# Autodesk Inventor assembly: Manipulator
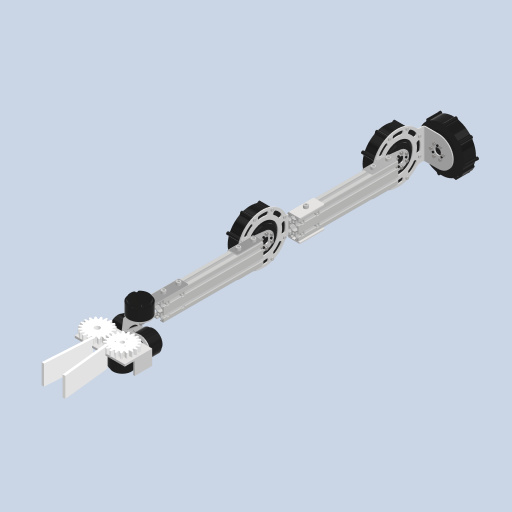
[picture p0: Inventor's stored thumbnail of the model, 512x512]
Saved by Autodesk Inventor 2023 (Build 270158000, 158)
## iProperties
Created: 2024-11-08
Part Number: Manipulator
Document SubType Name: Assembly
Designer: kiyo
Author: kiyo
## Documents named in this file (22)
- D:\GitHub\inventor\syu-si\OfficeRobot\Manipulator\Manipulator.iam
- D:\GitHub\inventor\syu-si\OfficeRobot\ReadyMade\Steadywin\GIM8108-8.iam
- D:\GitHub\inventor\syu-si\OfficeRobot\Manipulator\sholder-roll-bracket.ipt
- D:\GitHub\inventor\syu-si\OfficeRobot\Manipulator\elbow-pitch-bracket.ipt
- D:\GitHub\inventor\syu-si\OfficeRobot\Manipulator\Hand.iam
- D:\GitHub\inventor\syu-si\OfficeRobot\ReadyMade\Screw\M3_6mm.ipt
- D:\GitHub\inventor\syu-si\OfficeRobot\ReadyMade\Screw\SCB5-22.ipt
- D:\GitHub\inventor\syu-si\OfficeRobot\ReadyMade\Screw\HNTP5-5.ipt
- D:\GitHub\inventor\syu-si\OfficeRobot\Manipulator\pitch_plate_40mm.ipt
- D:\GitHub\inventor\syu-si\OfficeRobot\ReadyMade\Steadywin\GIM3505-8_with-driver.ipt
- D:\GitHub\inventor\syu-si\OfficeRobot\Manipulator\wrist_roll_plate.ipt
- D:\GitHub\inventor\syu-si\OfficeRobot\Manipulator\wrist-pitch-plate.ipt
- D:\GitHub\inventor\syu-si\OfficeRobot\Manipulator\wrist-yaw-plate.ipt
- D:\GitHub\inventor\syu-si\OfficeRobot\ReadyMade\Screw\M2-5_6mm.ipt
- D:\GitHub\inventor\syu-si\OfficeRobot\ReadyMade\Aluminum-frame\HFS5-2040-200-AV160-BV190-Z5-YA10-YB40.ipt
- D:\GitHub\inventor\syu-si\OfficeRobot\ReadyMade\Screw\SCB5-46.ipt
- D:\GitHub\inventor\syu-si\OfficeRobot\ReadyMade\Screw\SLBNR5.ipt
- D:\GitHub\inventor\syu-si\OfficeRobot\ReadyMade\Screw\CBSH3-8.ipt
- D:\GitHub\inventor\syu-si\OfficeRobot\ReadyMade\Screw\HNTT5-5.ipt
- D:\GitHub\inventor\syu-si\OfficeRobot\ReadyMade\Screw\SCB5-8.ipt
- D:\GitHub\inventor\syu-si\OfficeRobot\ReadyMade\Screw\FWSJJ-D5-V2_6-T4_5.ipt
- D:\GitHub\inventor\syu-si\OfficeRobot\ReadyMade\Screw\M2-5_10mm.ipt
## Components (108 placed, 21 different names)
1. elbow-pitch-bracket:1 — 挿入:180, 挿入:181, 挿入:234, 挿入:235, 挿入:256, 挿入:257, 挿入:268, 挿入:269, 挿入:270, 挿入:271, 挿入:272, 挿入:273, 挿入:274, 挿入:275, 挿入:295, 挿入:296, 挿入:299, 挿入:300
2. sholder-roll-bracket:1 — 挿入:1, 挿入:2, 挿入:3, 肩ヨー, 挿入:102, 挿入:103, 挿入:104, 挿入:105, 挿入:106, 挿入:107, 挿入:260, 挿入:261, 挿入:262, 挿入:263, 挿入:264, 挿入:265, 挿入:266, 挿入:267
3. pitch_plate_40mm:1 — 挿入:165, 挿入:182, 挿入:183, 挿入:184, 挿入:185, 挿入:186, 挿入:187, 挿入:232, 挿入:233, 角度:7, 挿入:250, 挿入:251, 挿入:254, 挿入:255, 挿入:278, 挿入:279, 角度:9, 角度:10
4. pitch_plate_40mm:2 — 挿入:190, 挿入:191, 挿入:192, 挿入:193, 挿入:194, 挿入:195, 挿入:196, 角度:8, 挿入:236, 挿入:237, 挿入:248, 挿入:249, 挿入:252, 挿入:253
5. wrist_roll_plate:1 — 挿入:220, 挿入:227, 挿入:228, 挿入:229, 挿入:230, 挿入:231, 挿入:283, 挿入:284, 挿入:285
6. wrist-pitch-plate:1 — 挿入:211, 挿入:212, 挿入:213, 挿入:217, 挿入:218, 挿入:219, 挿入:220, 挿入:280, 挿入:281, 挿入:282, 角度:15
7. wrist-yaw-plate:1 — 挿入:203, 挿入:204, 挿入:205, 挿入:206, 挿入:207, 挿入:211, 挿入:238, 挿入:239, 挿入:258, 挿入:259, 挿入:291, 挿入:292
8. HFS5-2040-200-AV160-BV190-Z5-YA10-YB40:1 — 挿入:232, 挿入:233, 挿入:234, 挿入:235, 挿入:246, 挿入:247, 挿入:293, 挿入:294, 角度:13, 角度:14
9. HFS5-2040-200-AV160-BV190-Z5-YA10-YB40:2 — 挿入:236, 挿入:237, 挿入:238, 挿入:239, 挿入:244, 挿入:245, 角度:11, 角度:12
10. Hand:1 [sub-assembly] — ハンド, 挿入:301
11. SCB5-22:1 — 挿入:247
12. SCB5-22:2 — 挿入:246
13. SCB5-22:3 — 挿入:244
14. SCB5-22:4 — 挿入:245
15. SCB5-46:1 — 挿入:250
16. SCB5-46:2 — 挿入:251
17. SCB5-46:3 — 挿入:248
18. SCB5-46:4 — 挿入:249
19. SLBNR5:1 — 挿入:255
20. SLBNR5:2 — 挿入:254
21. SLBNR5:3 — 挿入:252
22. SLBNR5:4 — 挿入:253
23. SLBNR5:5 — 挿入:256
24. SLBNR5:6 — 挿入:257
25. SLBNR5:7 — 挿入:258
26. SLBNR5:8 — 挿入:259
27. HNTT5-5:1 — 挿入:276, 角度:10
28. HNTT5-5:2 — 挿入:277, 角度:9
29. SCB5-8:1 — 挿入:276, 挿入:278
30. SCB5-8:2 — 挿入:277, 挿入:279
31. FWSJJ-D5-V2_6-T4_5:7 — 挿入:286
32. FWSJJ-D5-V2_6-T4_5:8 — 挿入:287
33. FWSJJ-D5-V2_6-T4_5:9 — 挿入:288
34. HNTT5-5:3 — 角度:11
35. HNTT5-5:4 — 角度:12
36. SCB5-8:3 — 挿入:291
37. SCB5-8:4 — 挿入:292
38. SCB5-22:5 — 挿入:294
39. SCB5-22:6 — 挿入:293
40. SLBNR5:9 — 挿入:296
41. SLBNR5:10 — 挿入:295
42. HNTT5-5:5 — 角度:13
43. SCB5-8:5 — 挿入:299
44. HNTT5-5:6 — 角度:14
45. SCB5-8:6 — 挿入:300
46. M3_6mm:1 — 挿入:183
47. M3_6mm:2 — 挿入:186
48. M3_6mm:3 — 挿入:187
49. M3_6mm:4 — 挿入:184
50. M3_6mm:5 — 挿入:185
51. M3_6mm:6 — 挿入:182
52. M3_6mm:7 — 挿入:192
53. M3_6mm:8 — 挿入:191
54. M3_6mm:9 — 挿入:196
55. M3_6mm:10 — 挿入:195
56. M3_6mm:11 — 挿入:194
57. M3_6mm:12 — 挿入:193
58. M3_6mm:13 — 挿入:107
59. M3_6mm:14 — 挿入:106
60. M3_6mm:15 — 挿入:105
61. M3_6mm:16 — 挿入:102
62. M3_6mm:17 — 挿入:103
63. M3_6mm:18 — 挿入:104
64. CBSH3-8:1 — 挿入:261
65. CBSH3-8:2 — 挿入:262
66. CBSH3-8:3 — 挿入:266
67. CBSH3-8:4 — 挿入:265
68. CBSH3-8:5 — 挿入:267
69. CBSH3-8:6 — 挿入:264
70. CBSH3-8:7 — 挿入:263
71. CBSH3-8:8 — 挿入:260
72. CBSH3-8:9 — 挿入:268
73. CBSH3-8:10 — 挿入:270
74. CBSH3-8:11 — 挿入:275
75. CBSH3-8:12 — 挿入:274
76. CBSH3-8:13 — 挿入:273
77. CBSH3-8:14 — 挿入:272
78. CBSH3-8:15 — 挿入:271
79. CBSH3-8:16 — 挿入:269
80. M2-5_6mm:1 — 挿入:205
81. M2-5_6mm:2 — 挿入:207
82. M2-5_6mm:3 — 挿入:206
83. M2-5_6mm:7 — 挿入:229
84. M2-5_6mm:8 — 挿入:230
85. M2-5_6mm:9 — 挿入:231
86. M2-5_6mm:4 — 挿入:217
87. M2-5_6mm:5 — 挿入:218
88. M2-5_6mm:6 — 挿入:219
89. M2-5_10mm:1
90. M2-5_10mm:2
91. M2-5_10mm:3
92. M2-5_10mm:4
93. M2-5_10mm:5
94. M2-5_10mm:6
95. FWSJJ-D5-V2_6-T4_5:1 — 挿入:280
96. FWSJJ-D5-V2_6-T4_5:2 — 挿入:282
97. FWSJJ-D5-V2_6-T4_5:3 — 挿入:281
98. FWSJJ-D5-V2_6-T4_5:4 — 挿入:283
99. FWSJJ-D5-V2_6-T4_5:5 — 挿入:285
100. FWSJJ-D5-V2_6-T4_5:6 — 挿入:284
101. HNTP5-5:7
102. HNTP5-5:8
103. GIM3505-8_with-driver:1 — 挿入:203, 挿入:204
104. GIM3505-8_with-driver:3 — 挿入:227, 挿入:228, 挿入:286, 挿入:287, 挿入:288, 角度:16, 挿入:301
105. GIM3505-8_with-driver:4 — 挿入:212, 挿入:213
106. GIM8108-8:1 [sub-assembly] — 挿入:1
107. GIM8108-8:2 [sub-assembly] — 挿入:2, 挿入:3, 挿入:165
108. GIM8108-8:3 [sub-assembly] — 挿入:180, 挿入:181, 挿入:190
## Relationships (126: Insert 114, Angle 12)
- 挿入:1 [Insert]: sholder-roll-bracket:1 ↔ GIM8108-8:1
- 挿入:2 [Insert]: sholder-roll-bracket:1 ↔ GIM8108-8:2
- 挿入:3 [Insert]: sholder-roll-bracket:1 ↔ GIM8108-8:2
- 肩ヨー [Angle] (0 deg): sholder-roll-bracket:1
- ハンド [Angle] (0 deg): Hand:1
- 挿入:102 [Insert]: sholder-roll-bracket:1 ↔ M3_6mm:16
- 挿入:103 [Insert]: sholder-roll-bracket:1 ↔ M3_6mm:17
- 挿入:104 [Insert]: sholder-roll-bracket:1 ↔ M3_6mm:18
- 挿入:105 [Insert]: sholder-roll-bracket:1 ↔ M3_6mm:15
- 挿入:106 [Insert]: sholder-roll-bracket:1 ↔ M3_6mm:14
- 挿入:107 [Insert]: sholder-roll-bracket:1 ↔ M3_6mm:13
- 挿入:165 [Insert]: pitch_plate_40mm:1 ↔ GIM8108-8:2
- 挿入:180 [Insert]: elbow-pitch-bracket:1 ↔ GIM8108-8:3
- 挿入:181 [Insert]: elbow-pitch-bracket:1 ↔ GIM8108-8:3
- 挿入:182 [Insert]: pitch_plate_40mm:1 ↔ M3_6mm:6
- 挿入:183 [Insert]: pitch_plate_40mm:1 ↔ M3_6mm:1
- 挿入:184 [Insert]: pitch_plate_40mm:1 ↔ M3_6mm:4
- 挿入:185 [Insert]: pitch_plate_40mm:1 ↔ M3_6mm:5
- 挿入:186 [Insert]: pitch_plate_40mm:1 ↔ M3_6mm:2
- 挿入:187 [Insert]: pitch_plate_40mm:1 ↔ M3_6mm:3
- 挿入:190 [Insert]: pitch_plate_40mm:2 ↔ GIM8108-8:3
- 挿入:191 [Insert]: pitch_plate_40mm:2 ↔ M3_6mm:8
- 挿入:192 [Insert]: pitch_plate_40mm:2 ↔ M3_6mm:7
- 挿入:193 [Insert]: pitch_plate_40mm:2 ↔ M3_6mm:12
- 挿入:194 [Insert]: pitch_plate_40mm:2 ↔ M3_6mm:11
- 挿入:195 [Insert]: pitch_plate_40mm:2 ↔ M3_6mm:10
- 挿入:196 [Insert]: pitch_plate_40mm:2 ↔ M3_6mm:9
- 挿入:203 [Insert]: wrist-yaw-plate:1 ↔ GIM3505-8_with-driver:1
- 挿入:204 [Insert]: wrist-yaw-plate:1 ↔ GIM3505-8_with-driver:1
- 挿入:205 [Insert]: wrist-yaw-plate:1 ↔ M2-5_6mm:1
- 挿入:206 [Insert]: wrist-yaw-plate:1 ↔ M2-5_6mm:3
- 挿入:207 [Insert]: wrist-yaw-plate:1 ↔ M2-5_6mm:2
- 挿入:211 [Insert] (3.5 mm): wrist-pitch-plate:1 ↔ wrist-yaw-plate:1
- 挿入:212 [Insert]: wrist-pitch-plate:1 ↔ GIM3505-8_with-driver:4
- 挿入:213 [Insert]: wrist-pitch-plate:1 ↔ GIM3505-8_with-driver:4
- 挿入:217 [Insert]: wrist-pitch-plate:1 ↔ M2-5_6mm:4
- 挿入:218 [Insert]: wrist-pitch-plate:1 ↔ M2-5_6mm:5
- 挿入:219 [Insert]: wrist-pitch-plate:1 ↔ M2-5_6mm:6
- 挿入:220 [Insert] (3.5 mm): wrist_roll_plate:1 ↔ wrist-pitch-plate:1
- [Insert]: wrist-pitch-plate:1 ↔ M2-5_10mm:1
- [Insert]: wrist-pitch-plate:1 ↔ M2-5_10mm:2
- [Insert]: wrist-pitch-plate:1 ↔ M2-5_10mm:3
- [Insert]: wrist_roll_plate:1 ↔ M2-5_10mm:6
- [Insert]: wrist_roll_plate:1 ↔ M2-5_10mm:4
- [Insert]: wrist_roll_plate:1 ↔ M2-5_10mm:5
- 挿入:227 [Insert]: wrist_roll_plate:1 ↔ GIM3505-8_with-driver:3
- 挿入:228 [Insert]: wrist_roll_plate:1 ↔ GIM3505-8_with-driver:3
- 挿入:229 [Insert]: wrist_roll_plate:1 ↔ M2-5_6mm:7
- 挿入:230 [Insert]: wrist_roll_plate:1 ↔ M2-5_6mm:8
- 挿入:231 [Insert]: wrist_roll_plate:1 ↔ M2-5_6mm:9
- 挿入:232 [Insert]: pitch_plate_40mm:1 ↔ HFS5-2040-200-AV160-BV190-Z5-YA10-YB40:1
- 挿入:233 [Insert]: pitch_plate_40mm:1 ↔ HFS5-2040-200-AV160-BV190-Z5-YA10-YB40:1
- 挿入:234 [Insert] (6 mm): elbow-pitch-bracket:1 ↔ HFS5-2040-200-AV160-BV190-Z5-YA10-YB40:1
- 挿入:235 [Insert] (6 mm): elbow-pitch-bracket:1 ↔ HFS5-2040-200-AV160-BV190-Z5-YA10-YB40:1
- 角度:7 [Angle] (0 deg): pitch_plate_40mm:1
- 角度:8 [Angle] (0 deg): pitch_plate_40mm:2
- 挿入:236 [Insert]: pitch_plate_40mm:2 ↔ HFS5-2040-200-AV160-BV190-Z5-YA10-YB40:2
- 挿入:237 [Insert]: pitch_plate_40mm:2 ↔ HFS5-2040-200-AV160-BV190-Z5-YA10-YB40:2
- 挿入:238 [Insert] (6 mm): wrist-yaw-plate:1 ↔ HFS5-2040-200-AV160-BV190-Z5-YA10-YB40:2
- 挿入:239 [Insert] (6 mm): wrist-yaw-plate:1 ↔ HFS5-2040-200-AV160-BV190-Z5-YA10-YB40:2
- 挿入:244 [Insert]: HFS5-2040-200-AV160-BV190-Z5-YA10-YB40:2 ↔ SCB5-22:3
- 挿入:245 [Insert]: HFS5-2040-200-AV160-BV190-Z5-YA10-YB40:2 ↔ SCB5-22:4
- 挿入:246 [Insert]: HFS5-2040-200-AV160-BV190-Z5-YA10-YB40:1 ↔ SCB5-22:2
- 挿入:247 [Insert]: HFS5-2040-200-AV160-BV190-Z5-YA10-YB40:1 ↔ SCB5-22:1
- 挿入:248 [Insert]: pitch_plate_40mm:2 ↔ SCB5-46:3
- 挿入:249 [Insert]: pitch_plate_40mm:2 ↔ SCB5-46:4
- 挿入:250 [Insert]: pitch_plate_40mm:1 ↔ SCB5-46:1
- 挿入:251 [Insert]: pitch_plate_40mm:1 ↔ SCB5-46:2
- 挿入:252 [Insert]: pitch_plate_40mm:2 ↔ SLBNR5:3
- 挿入:253 [Insert]: pitch_plate_40mm:2 ↔ SLBNR5:4
- 挿入:254 [Insert]: pitch_plate_40mm:1 ↔ SLBNR5:2
- 挿入:255 [Insert]: pitch_plate_40mm:1 ↔ SLBNR5:1
- 挿入:256 [Insert]: elbow-pitch-bracket:1 ↔ SLBNR5:5
- 挿入:257 [Insert]: elbow-pitch-bracket:1 ↔ SLBNR5:6
- 挿入:258 [Insert]: wrist-yaw-plate:1 ↔ SLBNR5:7
- 挿入:259 [Insert]: wrist-yaw-plate:1 ↔ SLBNR5:8
- 挿入:260 [Insert]: sholder-roll-bracket:1 ↔ CBSH3-8:8
- 挿入:261 [Insert]: sholder-roll-bracket:1 ↔ CBSH3-8:1
- 挿入:262 [Insert]: sholder-roll-bracket:1 ↔ CBSH3-8:2
- 挿入:263 [Insert]: sholder-roll-bracket:1 ↔ CBSH3-8:7
- 挿入:264 [Insert]: sholder-roll-bracket:1 ↔ CBSH3-8:6
- 挿入:265 [Insert]: sholder-roll-bracket:1 ↔ CBSH3-8:4
- 挿入:266 [Insert]: sholder-roll-bracket:1 ↔ CBSH3-8:3
- 挿入:267 [Insert]: sholder-roll-bracket:1 ↔ CBSH3-8:5
- 挿入:268 [Insert]: elbow-pitch-bracket:1 ↔ CBSH3-8:9
- 挿入:269 [Insert]: elbow-pitch-bracket:1 ↔ CBSH3-8:16
- 挿入:270 [Insert]: elbow-pitch-bracket:1 ↔ CBSH3-8:10
- 挿入:271 [Insert]: elbow-pitch-bracket:1 ↔ CBSH3-8:15
- 挿入:272 [Insert]: elbow-pitch-bracket:1 ↔ CBSH3-8:14
- 挿入:273 [Insert]: elbow-pitch-bracket:1 ↔ CBSH3-8:13
- 挿入:274 [Insert]: elbow-pitch-bracket:1 ↔ CBSH3-8:12
- 挿入:275 [Insert]: elbow-pitch-bracket:1 ↔ CBSH3-8:11
- 挿入:276 [Insert] (3.2 mm): HNTT5-5:1 ↔ SCB5-8:1
- 挿入:277 [Insert] (3.2 mm): HNTT5-5:2 ↔ SCB5-8:2
- 挿入:278 [Insert]: pitch_plate_40mm:1 ↔ SCB5-8:1
- 挿入:279 [Insert]: pitch_plate_40mm:1 ↔ SCB5-8:2
- 角度:9 [Angle] (0 deg): pitch_plate_40mm:1 ↔ HNTT5-5:2
- 角度:10 [Angle] (0 deg): pitch_plate_40mm:1 ↔ HNTT5-5:1
- 挿入:280 [Insert]: wrist-pitch-plate:1 ↔ FWSJJ-D5-V2_6-T4_5:1
- 挿入:281 [Insert]: wrist-pitch-plate:1 ↔ FWSJJ-D5-V2_6-T4_5:3
- 挿入:282 [Insert]: wrist-pitch-plate:1 ↔ FWSJJ-D5-V2_6-T4_5:2
- 挿入:283 [Insert]: wrist_roll_plate:1 ↔ FWSJJ-D5-V2_6-T4_5:4
- 挿入:284 [Insert]: wrist_roll_plate:1 ↔ FWSJJ-D5-V2_6-T4_5:6
- 挿入:285 [Insert]: wrist_roll_plate:1 ↔ FWSJJ-D5-V2_6-T4_5:5
- 挿入:286 [Insert]: FWSJJ-D5-V2_6-T4_5:7 ↔ GIM3505-8_with-driver:3
- 挿入:287 [Insert]: FWSJJ-D5-V2_6-T4_5:8 ↔ GIM3505-8_with-driver:3
- 挿入:288 [Insert]: FWSJJ-D5-V2_6-T4_5:9 ↔ GIM3505-8_with-driver:3
- [Insert] (3.2 mm): HNTT5-5:3 ↔ SCB5-8:3
- [Insert] (3.2 mm): HNTT5-5:4 ↔ SCB5-8:4
- 角度:11 [Angle] (0 deg): HFS5-2040-200-AV160-BV190-Z5-YA10-YB40:2 ↔ HNTT5-5:3
- 角度:12 [Angle] (0 deg): HFS5-2040-200-AV160-BV190-Z5-YA10-YB40:2 ↔ HNTT5-5:4
- 挿入:291 [Insert]: wrist-yaw-plate:1 ↔ SCB5-8:3
- 挿入:292 [Insert]: wrist-yaw-plate:1 ↔ SCB5-8:4
- 挿入:293 [Insert]: HFS5-2040-200-AV160-BV190-Z5-YA10-YB40:1 ↔ SCB5-22:6
- 挿入:294 [Insert]: HFS5-2040-200-AV160-BV190-Z5-YA10-YB40:1 ↔ SCB5-22:5
- 挿入:295 [Insert]: elbow-pitch-bracket:1 ↔ SLBNR5:10
- 挿入:296 [Insert]: elbow-pitch-bracket:1 ↔ SLBNR5:9
- [Insert] (3.2 mm): HNTT5-5:5 ↔ SCB5-8:5
- 角度:13 [Angle] (0 deg): HFS5-2040-200-AV160-BV190-Z5-YA10-YB40:1 ↔ HNTT5-5:5
- [Insert] (3.2 mm): HNTT5-5:6 ↔ SCB5-8:6
- 角度:14 [Angle] (0 deg): HFS5-2040-200-AV160-BV190-Z5-YA10-YB40:1 ↔ HNTT5-5:6
- 挿入:299 [Insert]: elbow-pitch-bracket:1 ↔ SCB5-8:5
- 挿入:300 [Insert]: elbow-pitch-bracket:1 ↔ SCB5-8:6
- 角度:15 [Angle] (90 deg): wrist-pitch-plate:1
- 角度:16 [Angle] (180 deg): GIM3505-8_with-driver:3
- 挿入:301 [Insert] (4.5 mm): Hand:1 ↔ GIM3505-8_with-driver:3
## Named parameters: d332_d317 = 3.2 mm, d333_d318 = 3.2 mm, d342_d317 = 3.2 mm, d344_d342_d317 = 3.2 mm
